# Autodesk Inventor assembly: 上層部
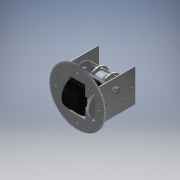
[picture p0: Inventor's stored thumbnail of the model, 180x180]
Saved by Autodesk Inventor 2019 (Build 230136000, 136)
## iProperties
Created: 2020-10-06
Part Number: 上層部
Material: 一般
Document SubType Name: Assembly
Designer: zhept
Mass: 1918.98 g
Surface Area: 3002 cm^2
Volume: 823.717 cm^3
Density: 2.32966 g/cm^3
Author: zhept
## Documents named in this file (19)
- C:\Users\zhept\OneDrive\大学\rrst\足回り2020\上層部\上層部.iam
- C:\Users\zhept\OneDrive\大学\rrst\足回り2020\上層部\板2.ipt
- C:\Users\zhept\OneDrive\大学\rrst\足回り2020\円柱5mm.ipt
- C:\Users\zhept\OneDrive\大学\rrst\足回り2020\足回り試作　ゴム車輪\モーター RS775-8513DF.iam
- C:\Users\zhept\OneDrive\大学\rrst\足回り2020\足回り試作　ゴム車輪\六角スペーサー.ipt
- C:\Users\zhept\OneDrive\大学\rrst\足回り2020\足回り試作　ゴム車輪\円 46.9mm.ipt
- C:\Users\zhept\OneDrive\大学\rrst\足回り2020\足回り試作　ゴム車輪\円 42.5mm.ipt
- C:\Users\zhept\OneDrive\大学\rrst\足回り2020\足回り試作　ゴム車輪\KHK_SS0530BOn.ipt
- C:\Users\zhept\OneDrive\大学\rrst\足回り2020\円柱8mm.ipt
- C:\Users\zhept\OneDrive\大学\rrst\足回り2020\KHK_SS05120AOn\KHK_SS05120AOn.ipt
- C:\Users\zhept\OneDrive\大学\rrst\足回り2020\HAMMER_CASTER_425ER100\HAMMER_CASTER_425ER100.ipt
- C:\Users\zhept\OneDrive\大学\rrst\足回り2020\KHK_SSG0840BOn\KHK_SSG0840BOn.ipt
- C:\Users\zhept\OneDrive\大学\rrst\足回り2020\KHK_SS08100AOn\KHK_SS08100AOn.ipt
- C:\Users\zhept\OneDrive\大学\rrst\足回り2020\IWATA_SCS0812CP3\SCS0812CP3.iam
- C:\Users\zhept\OneDrive\大学\rrst\足回り2020\足回り試作　ゴム車輪\板.ipt
- C:\Users\zhept\OneDrive\大学\rrst\足回り2020\金具 L型\金具 L型.ipt
- C:\Users\zhept\OneDrive\大学\rrst\足回り2020\KHK_SS2100J20On\SS2-100J20_On.ipt
- C:\Users\zhept\OneDrive\大学\rrst\玉軸受2 F608ZZ\玉軸受2 F608ZZ.ipt
- C:\Users\zhept\OneDrive\大学\rrst\足回り2020\IWATA_SCS0808CB2\SCS0808CB2.ipt
## Components (33 placed, 18 different names)
1. 板2:1 — メイト:2, 挿入:26, メイト:5, 挿入:35, 挿入:36, 挿入:37, 挿入:38, リジッド:3, リジッド:4
2. 円柱5mm:1 — 挿入:28
3. 円柱5mm:2 — 挿入:29
4. 円柱5mm:3 — 挿入:30
5. モーター RS775-8513DF:1 [sub-assembly] — 挿入:15
6. 六角スペーサー:1
7. 六角スペーサー:2
8. 円 46.9mm:1 — 挿入:9, 挿入:10, 挿入:11
9. 円 42.5mm:1 — 挿入:9, 挿入:10, 挿入:11
10. KHK_SS0530BOn:1 — 挿入:15, フラッシュ:1
11. 円柱8mm:1 — 円柱状:1, 円柱状:3
12. 円柱8mm:2 — 円柱状:2, 円柱状:4, 円柱状:5, 円柱状:6
13. KHK_SS05120AOn:1 — 円柱状:1, フラッシュ:1
14. HAMMER_CASTER_425ER100:1 — メイト:2, メイト:4
15. HAMMER_CASTER_425ER100:2 — 円柱状:2, メイト:3
16. KHK_SSG0840BOn:1 — 円柱状:3, フラッシュ:2
17. KHK_SS08100AOn:1 — 円柱状:4, フラッシュ:2, メイト:5
18. SCS0812CP3:1 [sub-assembly] — 円柱状:5, メイト:4
19. SCS0812CP3:2 [sub-assembly] — 円柱状:6, メイト:3
20. 板:1 — 挿入:26, 挿入:28, 挿入:29, 挿入:30, 挿入:31, 挿入:32, 挿入:33, 挿入:34, リジッド:1, リジッド:2
21. 金具 L型:1 — 挿入:31, 挿入:32, 挿入:39
22. 金具 L型:2 — 挿入:33, 挿入:34
23. 金具 L型:3 — 挿入:37, 挿入:38
24. 金具 L型:4 — 挿入:35, 挿入:36
25. SS2-100J20_On:1 — 挿入:39
26. SCS0808CB2:1 — メイト:9
27. SCS0808CB2:2 — メイト:8
28. SCS0808CB2:3 — メイト:7
29. SCS0808CB2:4 — メイト:6
30. 玉軸受2 F608ZZ:5 — リジッド:4, メイト:9
31. 玉軸受2 F608ZZ:6 — リジッド:3, メイト:8
32. 玉軸受2 F608ZZ:7 — リジッド:2, メイト:7
33. 玉軸受2 F608ZZ:8 — リジッド:1, メイト:6
## Relationships (41: Insert 17, Mate 9, CylindricalJoint 6, WeldJoint 4, RevoluteJoint 2, Flush 2, Angle 1)
- [RevoluteJoint]: モーター RS775-8513DF:1 ↔ 六角スペーサー:2
- [RevoluteJoint]: モーター RS775-8513DF:1 ↔ 六角スペーサー:1
- 挿入:9 [Insert] (40 mm): 円 46.9mm:1 ↔ 円 42.5mm:1
- 挿入:10 [Insert] (40 mm): 円 46.9mm:1 ↔ 円 42.5mm:1
- 挿入:11 [Insert] (40 mm): 円 46.9mm:1 ↔ 円 42.5mm:1
- 挿入:15 [Insert] (1 mm): モーター RS775-8513DF:1 ↔ KHK_SS0530BOn:1
- 円柱状:1 [CylindricalJoint]: 円柱8mm:1 ↔ KHK_SS05120AOn:1
- フラッシュ:1 [Flush]: KHK_SS0530BOn:1 ↔ KHK_SS05120AOn:1
- [Mate]: HAMMER_CASTER_425ER100:1 ↔ HAMMER_CASTER_425ER100:2
- [Angle] (0 deg): HAMMER_CASTER_425ER100:1 ↔ HAMMER_CASTER_425ER100:2
- 円柱状:2 [CylindricalJoint]: 円柱8mm:2 ↔ HAMMER_CASTER_425ER100:2
- メイト:2 [Mate] (65 mm): 板2:1 ↔ HAMMER_CASTER_425ER100:1
- 円柱状:3 [CylindricalJoint]: 円柱8mm:1 ↔ KHK_SSG0840BOn:1
- 円柱状:4 [CylindricalJoint]: 円柱8mm:2 ↔ KHK_SS08100AOn:1
- フラッシュ:2 [Flush]: KHK_SSG0840BOn:1 ↔ KHK_SS08100AOn:1
- 円柱状:5 [CylindricalJoint]: 円柱8mm:2 ↔ SCS0812CP3:1
- 円柱状:6 [CylindricalJoint]: 円柱8mm:2 ↔ SCS0812CP3:2
- メイト:3 [Mate]: HAMMER_CASTER_425ER100:2 ↔ SCS0812CP3:2
- メイト:4 [Mate]: HAMMER_CASTER_425ER100:1 ↔ SCS0812CP3:1
- 挿入:26 [Insert] (130 mm): 板2:1 ↔ 板:1
- 挿入:28 [Insert]: 円柱5mm:1 ↔ 板:1
- 挿入:29 [Insert]: 円柱5mm:2 ↔ 板:1
- 挿入:30 [Insert]: 円柱5mm:3 ↔ 板:1
- メイト:5 [Mate] (3 mm): 板2:1 ↔ KHK_SS08100AOn:1
- 挿入:31 [Insert]: 板:1 ↔ 金具 L型:1
- 挿入:32 [Insert]: 板:1 ↔ 金具 L型:1
- 挿入:33 [Insert]: 板:1 ↔ 金具 L型:2
- 挿入:34 [Insert]: 板:1 ↔ 金具 L型:2
- 挿入:35 [Insert]: 板2:1 ↔ 金具 L型:4
- 挿入:36 [Insert]: 板2:1 ↔ 金具 L型:4
- 挿入:37 [Insert]: 板2:1 ↔ 金具 L型:3
- 挿入:38 [Insert]: 板2:1 ↔ 金具 L型:3
- 挿入:39 [Insert]: 金具 L型:1 ↔ SS2-100J20_On:1
- リジッド:1 [WeldJoint]: 板:1 ↔ 玉軸受2 F608ZZ:8
- リジッド:2 [WeldJoint]: 板:1 ↔ 玉軸受2 F608ZZ:7
- リジッド:3 [WeldJoint]: 板2:1 ↔ 玉軸受2 F608ZZ:6
- リジッド:4 [WeldJoint]: 板2:1 ↔ 玉軸受2 F608ZZ:5
- メイト:6 [Mate]: SCS0808CB2:4 ↔ 玉軸受2 F608ZZ:8
- メイト:7 [Mate]: SCS0808CB2:3 ↔ 玉軸受2 F608ZZ:7
- メイト:8 [Mate]: SCS0808CB2:2 ↔ 玉軸受2 F608ZZ:6
- メイト:9 [Mate]: SCS0808CB2:1 ↔ 玉軸受2 F608ZZ:5
## Named parameters: d48_d46 = 0 mm, d49_d47 = 0 deg
